# Autodesk Inventor assembly: parts_combined_3D_Printer1
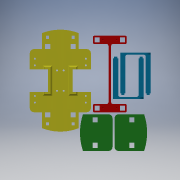
[picture p0: Inventor's stored thumbnail of the model, 180x180]
Saved by Autodesk Inventor 2016 (Build 200138000, 138)
## iProperties
Created: 2016-07-26
Part Number: parts_combined_3D_Printer1
Material: Générique
Document SubType Name: Assembly
Designer: tmonglon
Author: tmonglon
## Documents named in this file (5)
- D:\Inventor\Ahmet\AAA\chassis-nov2016\design\set1_to_print.iam
- D:\Inventor\Ahmet\AAA\chassis-nov2016\design\yellow_part.ipt
- D:\Inventor\Ahmet\AAA\chassis-nov2016\design\green_part.ipt
- D:\Inventor\Ahmet\AAA\chassis-nov2016\design\red_part.ipt
- D:\Inventor\Ahmet\AAA\chassis-nov2016\design\Blue_part.ipt
## Components (6 placed, 4 different names)
1. yellow_part:1 — Affleurement:1, Placage:1, Affleurement:4, Placage:4
2. green_part:1 — Affleurement:2, Placage:2, Affleurement:3, Placage:3
3. green_part:2 — Affleurement:1, Affleurement:2, Placage:1, Placage:2, Affleurement:3
4. red_part:1 — Affleurement:4, Placage:3, Placage:4, Affleurement:5, Placage:5, Placage:6
5. Blue_part:1 — Affleurement:5, Placage:5, Placage:6, Affleurement:6, Placage:7
6. Blue_part:2 — Affleurement:6, Placage:7
## Relationships (13: Mate 7, Flush 6)
- Affleurement:1 [Flush]: yellow_part:1 ↔ green_part:2
- Affleurement:2 [Flush]: green_part:1 ↔ green_part:2
- Placage:1 [Mate] (2 mm): yellow_part:1 ↔ green_part:2
- Placage:2 [Mate] (2 mm): green_part:1 ↔ green_part:2
- Affleurement:3 [Flush]: green_part:1 ↔ green_part:2
- Affleurement:4 [Flush]: yellow_part:1 ↔ red_part:1
- Placage:3 [Mate] (2 mm): green_part:1 ↔ red_part:1
- Placage:4 [Mate] (2 mm): yellow_part:1 ↔ red_part:1
- Affleurement:5 [Flush]: red_part:1 ↔ Blue_part:1
- Placage:5 [Mate] (2 mm): red_part:1 ↔ Blue_part:1
- Placage:6 [Mate] (5 mm): red_part:1 ↔ Blue_part:1
- Affleurement:6 [Flush]: Blue_part:1 ↔ Blue_part:2
- Placage:7 [Mate] (2 mm): Blue_part:1 ↔ Blue_part:2
